# Autodesk Inventor assembly: Shim_Assem_V3
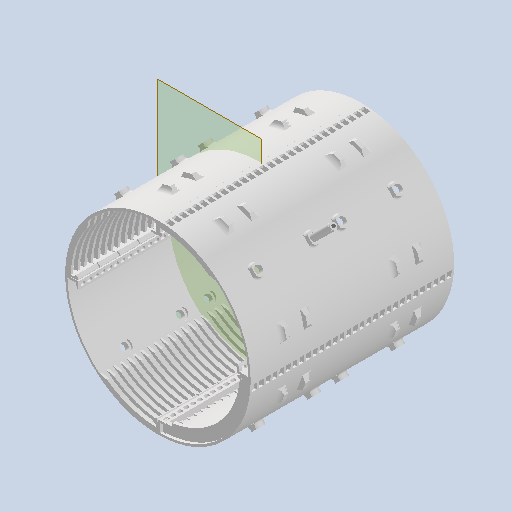
[picture p0: Inventor's stored thumbnail of the model, 512x512]
Saved by Autodesk Inventor 2025.2 (Build 292293000, 293)
## iProperties
Created: 2024-04-08
Part Number: Shim_Assem_V3
Document SubType Name: Assembly
Designer: Joshua Harper
Author: Joshua Harper
## Documents named in this file (4)
- C:\Users\Carla Fernandez\Documents\GitHub\OSII_MINI_V2\CAD MODELS\Shim_Assem_V4.iam
- C:\Users\Carla Fernandez\Documents\GitHub\OSII_MINI_V2\CAD MODELS\shim_tray_V4.ipt
- C:\Users\Carla Fernandez\Documents\GitHub\OSII_MINI_V2\CAD MODELS\shim_peg_V3.ipt
- C:\Users\Carla Fernandez\Documents\GitHub\OSII_MINI_V2\CAD MODELS\shim_cartridge_V3.ipt
## Components (6 placed, 3 different names)
1. shim_tray_V4:1 — Mate:1, Mate:2, Flush:1, Flush:3, Mate:7, Mate:8, Mate:9
2. shim_tray_V4:2 — Mate:1, Mate:2, Flush:1, Mate:3, Mate:4, Flush:2, Mate:10, Mate:11, Mate:12
3. shim_tray_V4:3 — Mate:3, Mate:4, Flush:2, Mate:5, Mate:6, Symmetry:1
4. shim_tray_V4:4 — Mate:5, Mate:6, Flush:3, Symmetry:1
5. shim_peg_V3:1 — Mate:10, Mate:11, Mate:12
6. shim_cartridge_V3:1 — Mate:7, Mate:8, Mate:9
## Relationships (16: Mate 12, Flush 3, Symmetry 1)
- Mate:1: shim_tray_V4:1 ↔ shim_tray_V4:2
- Mate:2: shim_tray_V4:1 ↔ shim_tray_V4:2
- Flush:1: shim_tray_V4:1 ↔ shim_tray_V4:2
- Mate:3: shim_tray_V4:2 ↔ shim_tray_V4:3
- Mate:4: shim_tray_V4:2 ↔ shim_tray_V4:3
- Flush:2: shim_tray_V4:2 ↔ shim_tray_V4:3
- Mate:5: shim_tray_V4:3 ↔ shim_tray_V4:4
- Mate:6: shim_tray_V4:3 ↔ shim_tray_V4:4
- Flush:3: shim_tray_V4:1 ↔ shim_tray_V4:4
- Mate:7: shim_tray_V4:1 ↔ shim_cartridge_V3:1
- Mate:8 (0.5 mm): shim_tray_V4:1 ↔ shim_cartridge_V3:1
- Mate:9: shim_tray_V4:1 ↔ shim_cartridge_V3:1
- Mate:10: shim_tray_V4:2 ↔ shim_peg_V3:1
- Mate:11: shim_tray_V4:2 ↔ shim_peg_V3:1
- Symmetry:1: shim_tray_V4:3 ↔ shim_tray_V4:4
- Mate:12: shim_tray_V4:2 ↔ shim_peg_V3:1
